# Autodesk Inventor assembly: drvassemblyrf
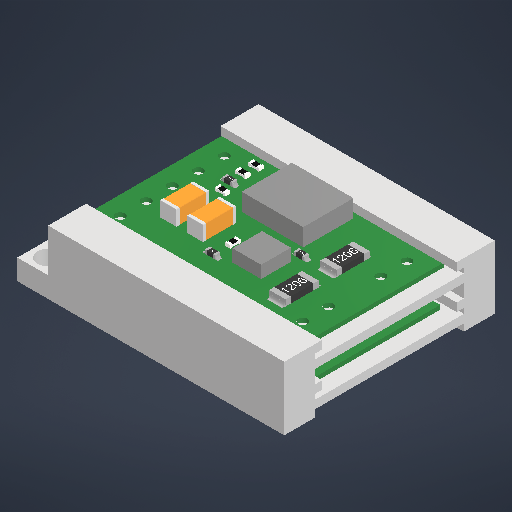
[picture p0: Inventor's stored thumbnail of the model, 512x512]
Saved by Autodesk Inventor 2026.2 (Build 302298010, 298A)
## iProperties
Created: 2026-05-11
Part Number: drvassemblyrf
Document SubType Name: Assembly
Designer: karol
Author: karol
## Documents named in this file (4)
- C:\Users\karol\OneDrive\Dokumenty\GitHub\bolt\bolt\cad\assembly\drvassemblyrf.iam
- drvassemblyrf.iam
- C:\Users\karol\OneDrive\Dokumenty\GitHub\bolt\bolt\cad\pcbs\drv\drv\drv.iam
- C:\Users\karol\OneDrive\Dokumenty\GitHub\bolt\bolt\cad\ready parts\drvholderlf.ipt
## Components (3 placed, 2 different names)
1. drvholderlf:1 — Mate:1, Mate:2, Flush:1, Mate:3, Mate:4, Flush:2
2. drv:1 [sub-assembly] — Mate:1, Mate:2, Flush:1
3. drv:2 [sub-assembly] — Mate:3, Mate:4, Flush:2
## Relationships (6: Mate 4, Flush 2)
- Mate:1: drvholderlf:1 ↔ drv:1
- Mate:2 (0.4 mm): drvholderlf:1 ↔ drv:1
- Flush:1: drvholderlf:1 ↔ drv:1
- Mate:3: drvholderlf:1 ↔ drv:2
- Mate:4: drvholderlf:1 ↔ drv:2
- Flush:2: drvholderlf:1 ↔ drv:2
